# Autodesk Inventor assembly: ASY MSC 600 cone exit back
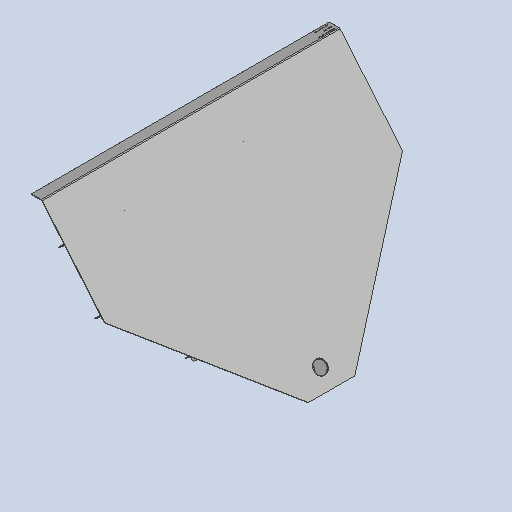
[picture p0: Inventor's stored thumbnail of the model, 512x512]
Saved by Autodesk Inventor 2025 (Build 290162010, 162A)
## iProperties
Created: 2024-08-26
Part Number: ASY MSC 600 cone exit back
Document SubType Name: Assembly
Designer: pokla
Stock Number: ASY МОО 600 конус выход корма
Author: pokla
## Documents named in this file (10)
- C:\Users\DELL\YandexDisk-badmisterfox\домашниий пк\Inventor\Manturovo\Manturovo_Se-clar\ASY MSC 600 cone exit back.iam
- C:\Users\DELL\YandexDisk-badmisterfox\домашниий пк\Inventor\Manturovo\Manturovo_Se-clar\MSC 601 cone exit back.ipt
- C:\Users\DELL\YandexDisk-badmisterfox\домашниий пк\Inventor\Manturovo\Manturovo_Se-clar\MSC 602 stringer cone exit back.ipt
- C:\Users\DELL\YandexDisk-badmisterfox\домашниий пк\Inventor\Manturovo\Manturovo_Se-clar\MSC 603 stringer cone exit back.ipt
- C:\Users\DELL\YandexDisk-badmisterfox\домашниий пк\Inventor\Manturovo\Manturovo_Se-clar\MSC 604 rib cone exit back.ipt
- C:\Users\DELL\YandexDisk-badmisterfox\домашниий пк\Inventor\Manturovo\Manturovo_Se-clar\MSC 605 rib cone exit back.ipt
- C:\Users\DELL\YandexDisk-badmisterfox\домашниий пк\Inventor\Manturovo\Manturovo_Se-clar\MSC 606 rocket tube 6.ipt
- C:\Users\DELL\YandexDisk-badmisterfox\домашниий пк\Inventor\Manturovo\Manturovo_Se-clar\MSC 607 rocket tube 7.ipt
- C:\Users\DELL\YandexDisk-badmisterfox\домашниий пк\Inventor\Manturovo\Manturovo_Se-clar\3d party\Stamp flange DIN2642\Stamd flange lapped collar DIN2642\Stamp flange DIN2642-065.ipt
- C:\Users\pokla\Documents\Inventor\Отстойник осветлитель\Manturovo_Se-clar-Gleb\Stamd flange lapped collar DIN2642.ipt
## Components (11 placed, 8 different names)
1. MSC 601 cone exit back:1 — Mate:5, Flush:1, Mate:6
2. MSC 602 stringer cone exit back:1 — Rigid:5, Rigid:11
3. MSC 602 stringer cone exit back:2 — Rigid:6
4. MSC 0162 stringer cone exit back:1 — Rigid:3, Rigid:10
5. MSC 0162 stringer cone exit back:2 — Rigid:4
6. MSC 0163 rib cone exit back:1 — Mate:5, Flush:1, Mate:6, Rigid:3, Rigid:4, Rigid:5, Rigid:6
7. MSC 0163 rib cone exit back:2 — Rigid:10
8. MSC 0164 rib cone exit back:1 — Rigid:11
9. MSC 606 rocket tube 6:1 — Rigid:9
10. MSC 607 rocket tube 7:1
11. Stamp flange DIN2642-065:1 — Rigid:9
## Relationships (12: WeldJoint 9, Mate 2, Flush 1)
- Mate:5: MSC 601 cone exit back:1 ↔ MSC 0163 rib cone exit back:1
- Flush:1: MSC 601 cone exit back:1 ↔ MSC 0163 rib cone exit back:1
- Mate:6 (200 mm): MSC 601 cone exit back:1 ↔ MSC 0163 rib cone exit back:1
- Rigid:3 [WeldJoint] (2 mm): MSC 0162 stringer cone exit back:1 ↔ MSC 0163 rib cone exit back:1
- Rigid:4 [WeldJoint] (2 mm): MSC 0162 stringer cone exit back:2 ↔ MSC 0163 rib cone exit back:1
- Rigid:5 [WeldJoint] (2 mm): MSC 602 stringer cone exit back:1 ↔ MSC 0163 rib cone exit back:1
- Rigid:6 [WeldJoint] (2 mm): MSC 602 stringer cone exit back:2 ↔ MSC 0163 rib cone exit back:1
- [WeldJoint]: MSC 601 cone exit back:1 ↔ MSC 607 rocket tube 7:1
- [WeldJoint]: MSC 606 rocket tube 6:1 ↔ MSC 607 rocket tube 7:1
- Rigid:9 [WeldJoint]: MSC 606 rocket tube 6:1 ↔ Stamp flange DIN2642-065:1
- Rigid:10 [WeldJoint] (2 mm): MSC 0162 stringer cone exit back:1 ↔ MSC 0163 rib cone exit back:2
- Rigid:11 [WeldJoint] (2 mm): MSC 602 stringer cone exit back:1 ↔ MSC 0164 rib cone exit back:1
